# Autodesk Inventor assembly: bumper
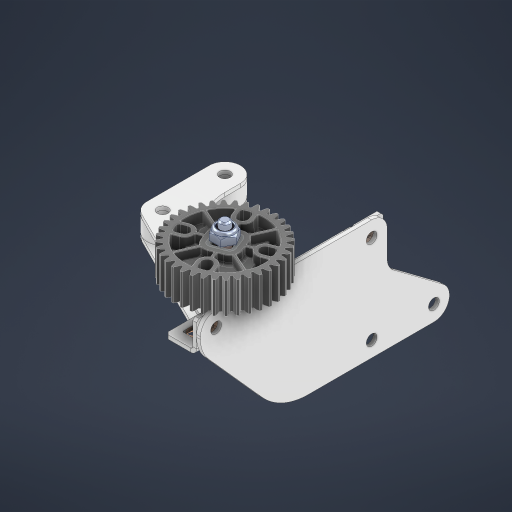
[picture p0: Inventor's stored thumbnail of the model, 512x512]
Saved by Autodesk Inventor 2024 (Build 280153000, 153)
## iProperties
Created: 2024-01-15
Part Number: bumper
Document SubType Name: Assembly
Designer: avere
Author: avere
## Documents named in this file (14)
- C:\Users\avere\Documents\rbp_cad\zoomba_v0.3\chassis\drivebay\bumper.iam
- C:\Users\avere\Documents\rbp_cad\zoomba_v0.3\chassis\drivebay\custom_parts\gusset.ipt
- C:\Users\avere\Documents\rbp_cad\VEX-CAD-Inventor-1.41\Motion\Spacers\Spacer Nylon .500 OD\NSpacer White .500 OD x .250.ipt
- C:\Users\avere\Documents\rbp_cad\VEX-CAD-Inventor-1.41\Motion\Spacers\Spacer Nylon .500 OD.ipt
- C:\Users\avere\Documents\rbp_cad\VEX-CAD-Inventor-1.41\Structure\Angle\Aluminum 1x1\Alu Angle 1x1x6.ipt
- C:\Users\avere\Documents\rbp_cad\zoomba_v0.3\chassis\drivebay\custom_parts\sled.ipt
- C:\Users\avere\Documents\rbp_cad\VEX-CAD-Inventor-1.41\Motion\Gears\HS Gear\HS 36T Gear, No Insert.iam
- C:\Users\avere\Documents\rbp_cad\VEX-CAD-Inventor-1.41\Motion\Gears\HS Gear.iam
- C:\Users\avere\Documents\rbp_cad\VEX-CAD-Inventor-1.41\Structure\Hardware\Screw Steel - Star\SScrew Star Smooth 1.750.ipt
- C:\Users\avere\Documents\rbp_cad\VEX-CAD-Inventor-1.41\Structure\Hardware\Screw Steel - Star.ipt
- C:\Users\avere\Documents\rbp_cad\VEX-CAD-Inventor-1.41\Structure\Hardware\Nut Keps.ipt
- C:\Users\avere\Documents\rbp_cad\VEX-CAD-Inventor-1.41\Motion\Spacers\Spacer Nylon .375 OD\NSpacer .375 OD x .375.ipt
- C:\Users\avere\Documents\rbp_cad\VEX-CAD-Inventor-1.41\Motion\Spacers\Spacer Nylon .375 OD.ipt
- C:\Users\avere\Documents\rbp_cad\VEX-CAD-Inventor-1.41\Structure\Hardware\Nut Thin Nylock.ipt
## Components (15 placed, 9 different names)
1. gusset:1 — Insert:1, Insert:2, Insert:5, Insert:7, Insert:9, Insert:14
2. gusset:2 — Insert:3, Insert:4, Insert:6, Insert:8, Insert:10, Insert:11, Mate:1
3. NSpacer White .500 OD x .250:1 — Insert:2, Insert:4
4. NSpacer White .500 OD x .250:2 — Insert:1, Insert:3
5. NSpacer White .500 OD x .250:3 — Insert:5, Insert:6
6. NSpacer White .500 OD x .250:4 — Insert:7, Insert:8
7. NSpacer White .500 OD x .250:5 — Insert:9
8. NSpacer White .500 OD x .250:6 — Insert:10
9. Alu Angle 1x1x6:1 — Insert:11, Mate:1, Insert:12, Mate:2, Insert:15
10. sled:1 — Insert:12, Mate:2
11. HS 36T Gear, No Insert:1 [sub-assembly] — Insert:17, Insert:18
12. SScrew Star Smooth 1.750:1 — Insert:14
13. Nut Keps:1 — Insert:15, Insert:16
14. NSpacer .375 OD x .375:1 — Insert:16, Insert:17
15. Nut Thin Nylock:1 — Insert:18
## Relationships (19: Insert 17, Mate 2)
- Insert:1: gusset:1 ↔ NSpacer White .500 OD x .250:2
- Insert:2: gusset:1 ↔ NSpacer White .500 OD x .250:1
- Insert:3: gusset:2 ↔ NSpacer White .500 OD x .250:2
- Insert:4: gusset:2 ↔ NSpacer White .500 OD x .250:1
- Insert:5: gusset:1 ↔ NSpacer White .500 OD x .250:3
- Insert:6: gusset:2 ↔ NSpacer White .500 OD x .250:3
- Insert:7: gusset:1 ↔ NSpacer White .500 OD x .250:4
- Insert:8: gusset:2 ↔ NSpacer White .500 OD x .250:4
- Insert:9: gusset:1 ↔ NSpacer White .500 OD x .250:5
- Insert:10: gusset:2 ↔ NSpacer White .500 OD x .250:6
- Insert:11: gusset:2 ↔ Alu Angle 1x1x6:1
- Mate:1: gusset:2 ↔ Alu Angle 1x1x6:1
- Insert:12: Alu Angle 1x1x6:1 ↔ sled:1
- Mate:2: Alu Angle 1x1x6:1 ↔ sled:1
- Insert:14: gusset:1 ↔ SScrew Star Smooth 1.750:1
- Insert:15: Alu Angle 1x1x6:1 ↔ Nut Keps:1
- Insert:16: Nut Keps:1 ↔ NSpacer .375 OD x .375:1
- Insert:17: HS 36T Gear, No Insert:1 ↔ NSpacer .375 OD x .375:1
- Insert:18 (0.3969 mm): HS 36T Gear, No Insert:1 ↔ Nut Thin Nylock:1
